# Autodesk Inventor assembly: Piston Assembly
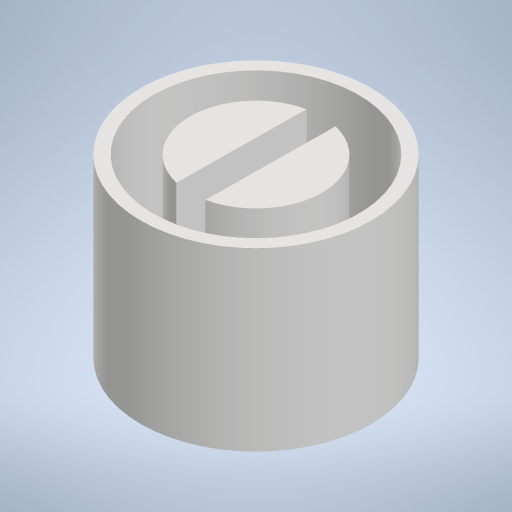
[picture p0: Inventor's stored thumbnail of the model, 512x512]
Saved by Autodesk Inventor 2023 (Build 270158000, 158)
## iProperties
Created: 2023-02-24
Part Number: Piston Assembly
Document SubType Name: Assembly
Designer: tommy
Author: tommy
## Documents named in this file (3)
- C:\Users\tommy\Documents\Repositories\Steam-Engine\Les Proper Steam Engine\CAD\Piston Assembly.iam
- C:\Users\tommy\Documents\Repositories\Steam-Engine\Les Proper Steam Engine\CAD\Piston Connector.ipt
- C:\Users\tommy\Documents\Repositories\Steam-Engine\Les Proper Steam Engine\CAD\Piston Crown.ipt
## Components (2 placed, 2 different names)
1. Piston Connector:1 — Mate:1, Mate:2
2. Piston Crown:1 — Mate:1, Mate:2
## Relationships (2: Mate 2)
- Mate:1: Piston Connector:1 ↔ Piston Crown:1
- Mate:2: Piston Connector:1 ↔ Piston Crown:1
